# Autodesk Inventor assembly: back_brace
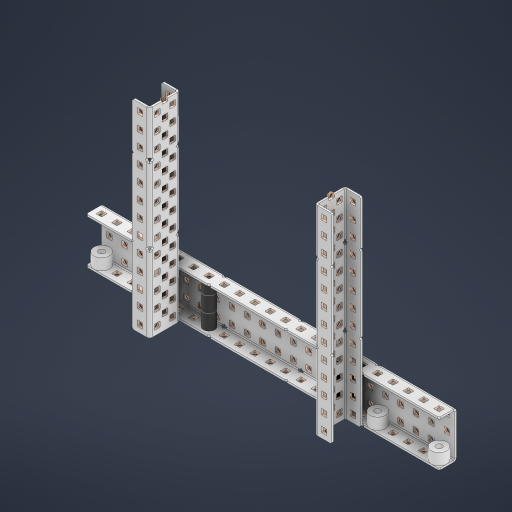
[picture p0: Inventor's stored thumbnail of the model, 512x512]
Saved by Autodesk Inventor 2024 (Build 280153000, 153)
## iProperties
Created: 2023-10-19
Part Number: back_brace
Document SubType Name: Assembly
Designer: avere
Author: avere
## Documents named in this file (8)
- C:\Users\avere\Documents\rbp_cad\goated_v0.1\chassis\back_brace.iam
- C:\Users\avere\Documents\rbp_cad\VEX-CAD-Inventor-1.41\Structure\C Channel\Aluminum 1x3x1\Alu C 1x3x1x23.ipt
- C:\Users\avere\Documents\rbp_cad\VEX-CAD-Inventor-1.41\Motion\Spacers\Spacer Nylon .375 OD\NSpacer .375 OD x .500.ipt
- C:\Users\avere\Documents\rbp_cad\VEX-CAD-Inventor-1.41\Motion\Spacers\Spacer Nylon .375 OD.ipt
- C:\Users\avere\Documents\rbp_cad\VEX-CAD-Inventor-1.41\Motion\Spacers\Spacer Nylon .375 OD\NSpacer .375 OD x .375.ipt
- C:\Users\avere\Documents\rbp_cad\VEX-CAD-Inventor-1.41\Motion\Spacers\Spacer Nylon .500 OD\NSpacer White .500 OD x .375.ipt
- C:\Users\avere\Documents\rbp_cad\VEX-CAD-Inventor-1.41\Motion\Spacers\Spacer Nylon .500 OD.ipt
- C:\Users\avere\Documents\rbp_cad\goated_v0.1\catapult\tower.iam
## Components (12 placed, 5 different names)
1. Alu C 1x3x1x23:1 — Insert:5, Insert:8, Insert:9, Insert:10, Insert:11, Insert:12, Insert:13, Mate:1
2. NSpacer .375 OD x .500:1 — Insert:4, Insert:5
3. NSpacer .375 OD x .500:2 — Insert:3, Insert:4
4. NSpacer .375 OD x .375:3 — Insert:3
5. NSpacer .375 OD x .500:4 — Insert:8
6. NSpacer .375 OD x .500:5
7. NSpacer .375 OD x .375:6
8. NSpacer White .500 OD x .375:1 — Insert:10
9. NSpacer White .500 OD x .375:2 — Insert:12
10. NSpacer White .500 OD x .375:3 — Insert:11
11. NSpacer White .500 OD x .375:4 — Insert:9
12. tower:1 [sub-assembly] — Insert:13, Mate:1
## Relationships (12: Insert 11, Mate 1)
- Insert:3: NSpacer .375 OD x .500:2 ↔ NSpacer .375 OD x .375:3
- Insert:4: NSpacer .375 OD x .500:1 ↔ NSpacer .375 OD x .500:2
- Insert:5: Alu C 1x3x1x23:1 ↔ NSpacer .375 OD x .500:1
- [Insert]: NSpacer .375 OD x .500:5 ↔ NSpacer .375 OD x .375:6
- [Insert]: NSpacer .375 OD x .500:4 ↔ NSpacer .375 OD x .500:5
- Insert:8: Alu C 1x3x1x23:1 ↔ NSpacer .375 OD x .500:4
- Insert:9: Alu C 1x3x1x23:1 ↔ NSpacer White .500 OD x .375:4
- Insert:10: Alu C 1x3x1x23:1 ↔ NSpacer White .500 OD x .375:1
- Insert:11: Alu C 1x3x1x23:1 ↔ NSpacer White .500 OD x .375:3
- Insert:12: Alu C 1x3x1x23:1 ↔ NSpacer White .500 OD x .375:2
- Insert:13 (12.7 mm): Alu C 1x3x1x23:1 ↔ tower:1
- Mate:1: Alu C 1x3x1x23:1 ↔ tower:1
## Named parameters: d5_d2 = 0 mm, d6_d3 = 0 mm
